# Autodesk Inventor assembly: Guardrail
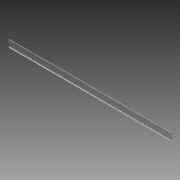
[picture p0: Inventor's stored thumbnail of the model, 180x180]
Saved by Autodesk Inventor 2013 (Build 170138000, 138)
## iProperties
Created: 2013-01-07
Part Number: Guardrail
Document SubType Name: Assembly
Designer: Phillip
_SolveAssemblyDoc: Frame Generator Solve Assembly
_Version: 15.0.0
Author: Phillip
## Documents named in this file (4)
- C:\Users\Moses\Documents\Inventor\2013 Team 3061 Robot\FIRST Arena 2013\Arena\Guardrail.iam
- C:\Users\Moses\Documents\Inventor\2013 Team 3061 Robot\FIRST Arena 2013\Arena\GuardrailFrame.ipt
- C:\Users\Moses\Documents\Inventor\2013 Team 3061 Robot\FIRST Arena 2013\Arena\Guardrail\Frame\Frame0001.iam
- C:\Users\Moses\Documents\Inventor\2013 Team 3061 Robot\FIRST Arena 2013\Arena\GuardShield.ipt
## Components (3 placed, 3 different names)
1. GuardrailFrame:1
2. Frame0001:1 [sub-assembly] — Flush:1, Flush:2
3. GuardShield:1 — Flush:1, Flush:2
## Relationships (2: Flush 2)
- Flush:1: Frame0001:1 ↔ GuardShield:1
- Flush:2: Frame0001:1 ↔ GuardShield:1
